# Autodesk Inventor assembly: RM/8010/M/50(Magnetic Piston,0,B,0)
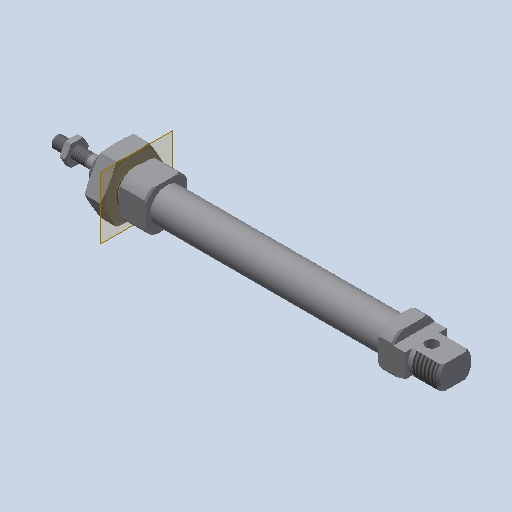
[picture p0: Inventor's stored thumbnail of the model, 512x512]
Saved by Autodesk Inventor 2026.1 (Build 301233000, 233)
## iProperties
Created: 2018-09-27
Part Number: RM/8010/M/50(Magnetic Piston,0,B,0)
Catalog Web Link: www.cadenas.de
Description: Series RM/8000/M + Mountings and Accessories-Roundline cylinder
Vendor: IMI
Document SubType Name: Assembly
Designer: psadmin
Manufacturer: IMI
Category: PARTsolutions
Company: IMI
PSOL_IDENT_0: {$CADENAS_DATA\23d-libs\imi_precision\1_actuators\1_roundline_cylinders\series_rm_8000_var_asmtab.pr
PSOL_IDENT_1: j},296 {VTYP=3D},{STYP=ASSTAB},{NB=RM/8010/M/50(Magnetic Piston,0,B,0)},{LINA=RM/8010/M/50},{NN=Seri
PSOL_IDENT_2: es RM/8000/M + Mountings and Accessories},{DATE=04.09.2018 05:58:30},{GEOMDATE=27.06.2018 08:21:58},
PSOL_IDENT_3: {VERSION=},{LINEID=10},{WBVAR=CH,BS,HUB,HRS,P,VAR,PR,FM,RM,RPR,S,PMU,HUBST},{WBNUMERIC=HUB,PMU,HUBST
PSOL_IDENT_4: }  {NB=RM/8010/M/50(Magnetic Piston,0,B,0)},{LINA=RM/8010/M/50},{KT=DUMMY},{CNSORDERNO=RM/8010/M/50}
PSOL_IDENT_5: ,{CH=B},{BS=010},{DALG=  '010' , '10' ,  '012' , '12'  ,  '016' , '16' ,  '020' , '20' ,  '025' , '2
PSOL_IDENT_6: 5'  },{HUB=50},{HUBALG=10,25,40,50,80,100,[5:500]},{HRS=},{HRSALG= '' ,  'Standard (pneumatic)'  },{
PSOL_IDENT_7: P=Magnetic Piston},{PX=  'Magnetic Piston' , 'Magnetic Piston'  , 'Non-Magnetic Piston' , 'Non-Magne
PSOL_IDENT_8: tic Piston' },{VAR=M},{VARALG=    'M' , 'M - Standard with integral eye mounting, no variant' , 'rm_
PSOL_IDENT_9: 8000_m.jpg'  ,  'MC' , 'MC - Central rear port' ,  'rm_8000_m.jpg' ,  'MF' , 'MF - Flat rear cover'
PSOL_IDENT_10: , 'rm_8000_m.jpg'  , 'MU' , 'MU - Extended piston rod'  , 'rm_8000_mu.jpg'   },{PR=},{PRALG= '' , 'N
PSOL_IDENT_11: one' , 'none.jpg' , '+QM/8010/38' , 'AK - Piston rod swivel' , 'ak.jpg' , '+QM/8010/25' , 'F - Pisto
PSOL_IDENT_12: n rod clevis' , 'f.jpg' , '+QM/8010/32' , 'UF - Piston rod eye' , 'uf.jpg' },{FM=},{FMALG= '' , 'Non
PSOL_IDENT_13: e' , 'none_fm.jpg' , '+M/P19369' , 'C - Foot Mounting', 'c.jpg' , '+M/P19407' , 'B/G - Front/rear fl
PSOL_IDENT_14: ange' , 'g_b.jpg'  },{RM=},{RMALG= '' , 'None' , 'none_rm.jpg' , '+M/P19369' , 'C - Foot Mounting' ,
PSOL_IDENT_15: 'c.jpg' , '+M/P19407' , 'B/G - Front/rear flange' , 'g_b.jpg' , '+QM/947' , 'L - Rear hinge' , 'l.j
PSOL_IDENT_16: pg' , '+QM/8010/44' , 'L2 - Rear hinge' , 'l2.jpg' , '+M/P1501/90' , 'N - Nut' , 'n.jpg' },{RPR=},{R
PSOL_IDENT_17: PRALG= '' , '-' , 'none.jpg'},{S=},{SALG= '' , 'None' , '+M/50/IOP/5V+QM/33/010/23'  , 'Solid state
PSOL_IDENT_18: switch with IO-Link mode and 5m cable'  , '+M/50/IOP/CP+QM/33/010/23'  , 'Solid state switch with IO
PSOL_IDENT_19: -Link mode and M8 connector' ,'+M/50/LSU/2V+QM/33/010/23'  , 'Reed switch with integral 2m PVC cable'
PSOL_IDENT_20: , '+M/50/LSU/5V+QM/33/010/23'  , 'Reed switch with integral 5m PVC cable'   , '+M/50/LSU/10V+QM/3
PSOL_IDENT_21: 3/010/23' , 'Reed switch with integral 10m PVC cable'  , '+M/50/LSU/5U+QM/33/010/23'  , 'Reed switch
PSOL_IDENT_22: with integral 5m PUR cable'   , '+TM/50/RAU/2S+QM/33/010/23' , 'Reed switch with integral 2m Silico
PSOL_IDENT_23: n cable'  , '+M/50/RAC/5V+QM/33/010/23'  , 'Reed switch with integral 5m PVC cable and changeover'
PSOL_IDENT_24: , '+M/50/LSU/CP+QM/33/010/23'  , 'Reed switch for plug-in cable M8x1'   , '+M/50/EAP/2V+QM/33/010/23'
PSOL_IDENT_25: , 'Solid state switch with integral 2m cable PNP'   , '+M/50/EAP/5V+QM/33/010/23'  , 'Solid state
PSOL_IDENT_26: switch with integral 5m cable PNP'   , '+M/50/EAP/10V+QM/33/010/23' , 'Solid state switch with integ
PSOL_IDENT_27: ral 10m cable PNP'  , '+M/50/EAP/5U+QM/33/010/23'  , 'Solid state switch with integral 5m PUR cable'
PSOL_IDENT_28: , '+M/50/EAP/CP+QM/33/010/23'  , 'Solid state switch for plug-in cable PNP M8x1'   ,'+M/50/EAP/CC
PSOL_IDENT_29: +QM/33/010/23'  , 'Solid state switch for plug-in cable PNP M12x1'  ,'+M/50/EAN/2V+QM/33/010/23'  , '
PSOL_IDENT_30: Solid state switch with integral 2m cable NPN'   , '+M/50/EAN/5V+QM/33/010/23'  , 'Solid state switc
PSOL_IDENT_31: h with integral 5m cable NPN'   , '+M/50/EAN/10V+QM/33/010/23' , 'Solid state switch with integral 1
PSOL_IDENT_32: 0m cable NPN'  , '+M/50/EAN/CP+QM/33/010/23'  , 'Solid state switch for plug-in cable NPN M8x1'    ,
PSOL_IDENT_33: '+M/50/IOP/5V+M/50/IOP/5V+QM/33/010/23'  , '2 x Solid state switch with IO-Link mode and 5m cable'
PSOL_IDENT_34: , '+M/50/IOP/CP+M/50/IOP/CP+QM/33/010/23'  , '2 x Solid state switch with IO-Link mode and M8 conne
PSOL_IDENT_35: ctor'   ,'+M/50/LSU/2V+M/50/LSU/2V+QM/33/010/23'  , '2 x Reed switch with integral 2m PVC cable'   ,
PSOL_IDENT_36: '+M/50/LSU/5V+M/50/LSU/5V+QM/33/010/23'  , '2 x Reed switch with integral 5m PVC cable'   , '+M/50/
PSOL_IDENT_37: LSU/10V+M/50/LSU/10V+QM/33/010/23' , '2 x Reed switch with integral 10m PVC cable'  , '+M/50/LSU/5U+
PSOL_IDENT_38: M/50/LSU/5U+QM/33/010/23'  , '2 x Reed switch with integral 5m PUR cable'   , '+TM/50/RAU/2S+TM/50/R
PSOL_IDENT_39: AU/2S+QM/33/010/23' , '2 x Reed switch with integral 2m Silicon cable'  , '+M/50/RAC/5V+M/50/RAC/5V+
PSOL_IDENT_40: QM/33/010/23'  , '2 x Reed switch with integral 5m PVC cable and changeover'  , '+M/50/LSU/CP+M/50/L
PSOL_IDENT_41: SU/CP+QM/33/010/23'  , '2 x Reed switch for plug-in cable M8x1'   , '+M/50/EAP/2V+M/50/EAP/2V+QM/33/
PSOL_IDENT_42: 010/23'  , '2 x Solid state switch with integral 2m cable PNP'   , '+M/50/EAP/5V+M/50/EAP/5V+QM/33/0
PSOL_IDENT_43: 10/23'  , '2 x Solid state switch with integral 5m cable PNP'   , '+M/50/EAP/10V+M/50/EAP/10V+QM/33/
PSOL_IDENT_44: 010/23' , '2 x Solid state switch with integral 10m cable PNP'  , '+M/50/EAP/5U+M/50/EAP/5U+QM/33/01
PSOL_IDENT_45: 0/23'  , '2 x Solid state switch with integral 5m PUR cable'   , '+M/50/EAP/CP+M/50/EAP/CP+QM/33/010
PSOL_IDENT_46: /23'  , '2 x Solid state switch for plug-in cable PNP M8x1'   ,'+M/50/EAP/CC+M/50/EAP/CC+QM/33/010/2
PSOL_IDENT_47: 3'  , '2 x Solid state switch for plug-in cable PNP M12x1'  ,'+M/50/EAN/2V+M/50/EAN/2V+QM/33/010/23'
PSOL_IDENT_48: , '2 x Solid state switch with integral 2m cable NPN'   , '+M/50/EAN/5V+M/50/EAN/5V+QM/33/010/23'
PSOL_IDENT_49: , '2 x Solid state switch with integral 5m cable NPN'   , '+M/50/EAN/10V+M/50/EAN/10V+QM/33/010/23'
PSOL_IDENT_50: , '2 x Solid state switch with integral 10m cable NPN'  , '+M/50/EAN/CP+M/50/EAN/CP+QM/33/010/23'
PSOL_IDENT_51: , '2 x Solid state switch for plug-in cable NPN M8x1'   },{PMU=0},{PMUALG=0},{HUBST=0},{INFOWWW=Link
PSOL_IDENT_52: },{AM=12},{B=12},{BA=12},{BE=M12x1.25},{BF=12},{CD=4},{D=16.5},{EE=M5},{EW=7.9},{G=9.0},{KK=M4},{KV=
PSOL_IDENT_53: 19},{KW=6},{KW1=2},{L=6},{L12=0},{LB=2},{MM=4},{MR=8},{PL=5.5},{KV1=7},{KV2=0},{KV4=14},{WF=16},{VA=
PSOL_IDENT_54: 1.5},{VD=1.5},{XC=64},{INFOPATH=http://cdn.norgren.com/pdf/en_1_5_041_RT_57200_M_RM_57200_M.pdf},{PP
PSOL_IDENT_55: ATH=assemblies/series_rm_8000_m2_asmtpl.prj},{TRANS1=N2 - Non-rotating piston rod},{TRANS2=L4 - Lock
PSOL_IDENT_56: ing unit},{TRANS3=61 - Guide block roller bearings},{RMO=}
NN: Series RM/8000/M + Mountings and Accessories
NT: Roundline cylinder
NB: RM/8010/M/50(Magnetic Piston,0,B,0)
NBSYN: $CNSORDERNO.($P.,$HUBST.,$CH.,$PMU.)
LINA: RM/8010/M/50
CNSORDERNO: RM/8010/M/50
CH: Buffer
BS: 10
HUB: 50
HRS: Standard
P: Magnetic Piston
VAR: M - Standard
RPR: -
PMU: 0
INFOWWW: Product Datasheet (PDF)
SUPPLIER: IMI
ARTICLENO: RM/8010/M/50(Magnetic Piston,0,B,0)
BOMINFO: RM/8010/M/50
CREATOR: CADENAS GmbH
Title: RM/8010/M/50
Author: Cadenas PARTsolutions
Comments: Roundline cylinder
## Documents named in this file (5)
- C:\Users\user\Desktop\setup_inventor_2025\Verbinder_Tisch_Dewar\IMI_PRECISION_RM8010M50MagneticPiston0B0\AIS2018\RM_8010_M_50(Magnetic Piston,0,B,0).iam
- C:\Users\user\Desktop\setup_inventor_2025\Verbinder_Tisch_Dewar\IMI_PRECISION_RM8010M50MagneticPiston0B0\AIS2018\RM_8010_M_50_B0__B.ipt
- C:\Users\user\Desktop\setup_inventor_2025\Verbinder_Tisch_Dewar\IMI_PRECISION_RM8010M50MagneticPiston0B0\AIS2018\RM_8010_N.ipt
- C:\Users\user\Desktop\setup_inventor_2025\Verbinder_Tisch_Dewar\IMI_PRECISION_RM8010M50MagneticPiston0B0\AIS2018\RM_8010_M_50_0_0_P.ipt
- C:\Users\user\Desktop\setup_inventor_2025\Verbinder_Tisch_Dewar\IMI_PRECISION_RM8010M50MagneticPiston0B0\AIS2018\RM_8010_N2.ipt
## Components (4 placed, 4 different names)
1. RM_8010_M_50_B0__B:1 — Symmetry:1
2. RM_8010_N:1 — Symmetry:1
3. RM_8010_M_50_0_0_P:1
4. RM_8010_N2:1
## Relationships (1: Symmetry 1)
- Symmetry:1: RM_8010_M_50_B0__B:1 ↔ RM_8010_N:1
